# Autodesk Inventor assembly: arm one
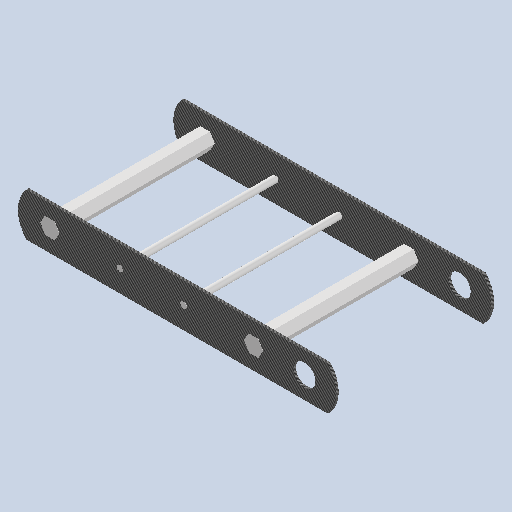
[picture p0: Inventor's stored thumbnail of the model, 512x512]
Saved by Autodesk Inventor 2023 (Build 270158000, 158)
## iProperties
Created: 2023-01-03
Part Number: arm one
Document SubType Name: Assembly
Designer: victo
Author: victo
## Documents named in this file (4)
- C:\Users\victo\OneDrive\Documents\rcr\completely new\arm one.iam
- C:\Users\victo\OneDrive\Documents\rcr\completely new\new arm plate.ipt
- C:\Users\victo\OneDrive\Documents\rcr\completely new\hex shaft.ipt
- C:\Users\victo\OneDrive\Documents\rcr\completely new\new rotary shaft.ipt
## Components (6 placed, 3 different names)
1. new arm plate:1 — Rigid:1, Rigid:3, Rotational:1, Rotational:2
2. new arm plate:2 — Rigid:2
3. hex shaft:1 — Rigid:1, Rigid:2
4. hex shaft:2 — Rigid:3
5. new rotary shaft:1 — Rotational:1
6. new rotary shaft:2 — Rotational:2
## Relationships (5: WeldJoint 3, RevoluteJoint 2)
- Rigid:1 [WeldJoint]: new arm plate:1 ↔ hex shaft:1
- Rigid:2 [WeldJoint]: new arm plate:2 ↔ hex shaft:1
- Rigid:3 [WeldJoint]: new arm plate:1 ↔ hex shaft:2
- Rotational:1 [RevoluteJoint]: new arm plate:1 ↔ new rotary shaft:1
- Rotational:2 [RevoluteJoint]: new arm plate:1 ↔ new rotary shaft:2
